# Autodesk Inventor assembly: Assembly1
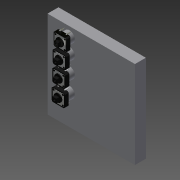
[picture p0: Inventor's stored thumbnail of the model, 180x180]
Saved by Autodesk Inventor 2019 (Build 230136000, 136)
## iProperties
Created: 2020-02-20
Part Number: Assembly1
Document SubType Name: Assembly
Designer: kaif alam
Author: kaif alam
## Documents named in this file (3)
- C:\Users\kaif alam\Documents\Assembly1.iam
- C:\Users\kaif alam\Documents\expwork.ipt
- C:\Users\kaif alam\Documents\KAN-1210.ipt
## Components (5 placed, 2 different names)
1. expwork:1 — Mate:1, Mate:2, Mate:3, Mate:4
2. KAN-1210:1 — Mate:1
3. KAN-1210:2 — Mate:3
4. KAN-1210:3 — Mate:4
5. KAN-1210:4 — Mate:2
## Relationships (4: Mate 4)
- Mate:1: expwork:1 ↔ KAN-1210:1
- Mate:2: expwork:1 ↔ KAN-1210:4
- Mate:3: expwork:1 ↔ KAN-1210:2
- Mate:4: expwork:1 ↔ KAN-1210:3
